# Autodesk Inventor assembly: ASSEMBLY_Y_axis_linear_shaft_mount
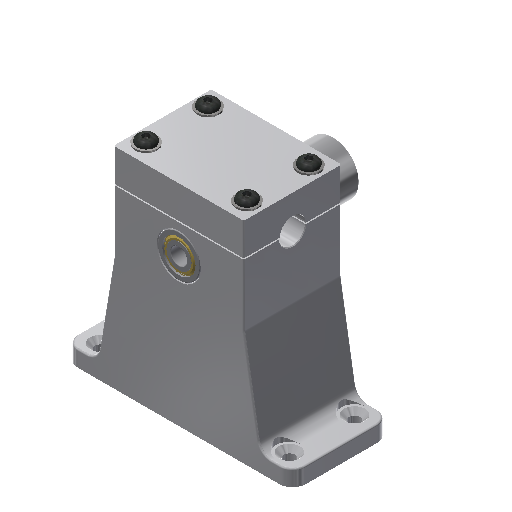
[picture p0: Inventor's stored thumbnail of the model, 512x512]
Saved by Autodesk Inventor 2026.1 (Build 301233000, 233)
## iProperties
Created: 2018-07-31
Part Number: ASSEMBLY_Y_axis_linear_shaft_mount
Document SubType Name: Assembly
Designer: Andrzej
Author: Andrzej
## Documents named in this file (8)
- C:\Users\Andrzej\OneDrive\_DRIVE_SYNCH_FILES\__ BYTECHLAB PROJECTS\MLTDIS - SMD Parts Sorting Machine\MCAD\1_REV1\ASSEMBLY_XY_AXIS_REVA\ASSEMBLY_Y_axis_linear_shaft_mount.iam
- C:\Users\Andrzej\OneDrive\_DRIVE_SYNCH_FILES\__ BYTECHLAB PROJECTS\MLTDIS - SMD Parts Sorting Machine\MCAD\1_REV1\ASSEMBLY_XY_AXIS_REVA\3DP_PLA_Y_axis_linear_shaft_mount_clamp.ipt
- C:\Users\Andrzej\OneDrive\_DRIVE_SYNCH_FILES\__ BYTECHLAB PROJECTS\MLTDIS - SMD Parts Sorting Machine\MCAD\1_REV1\ASSEMBLY_XY_AXIS_REVA\3DP_PLA_Y_axis_linear_shaft_mount.ipt
- C:\Users\Andrzej\OneDrive\_DRIVE_SYNCH_FILES\__ BYTECHLAB PROJECTS\MLTDIS - SMD Parts Sorting Machine\MCAD\1_REV1\__COTS_PARTS\COTS_AST_695HZZ_Bearing.ipt
- C:\Users\Andrzej\OneDrive\_DRIVE_SYNCH_FILES\__ BYTECHLAB PROJECTS\MLTDIS - SMD Parts Sorting Machine\MCAD\1_REV1\__COTS_PARTS\COTS_GENERIC_GT2_20T_Pulley.ipt
- C:\Users\Andrzej\OneDrive\_DRIVE_SYNCH_FILES\__ BYTECHLAB PROJECTS\MLTDIS - SMD Parts Sorting Machine\MCAD\1_REV1\ASSEMBLY_XY_AXIS_REVA\3DP_PLA_Y_axis_drive_shaft_pulley_washer.ipt
- C:\Users\Andrzej\OneDrive\_DRIVE_SYNCH_FILES\__ BYTECHLAB PROJECTS\MLTDIS - SMD Parts Sorting Machine\MCAD\1_REV1\__CONTENT_CENTER_PARTS\en-US\DIN 125-2  A\DIN 125-2 - A 3,2A.ipt
- C:\Users\Andrzej\OneDrive\_DRIVE_SYNCH_FILES\__ BYTECHLAB PROJECTS\MLTDIS - SMD Parts Sorting Machine\MCAD\1_REV1\__CONTENT_CENTER_PARTS\en-US\ISO 7380-1\ISO 7380-1 - M3 x 30.ipt
## Components (14 placed, 7 different names)
1. 3DP_PLA_Y_axis_linear_shaft_mount_clamp:1 — Mate:1, Flush:1, Flush:2, Insert:1, Insert:2, Insert:3, Insert:4
2. 3DP_PLA_Y_axis_linear_shaft_mount:1 — Mate:1, Flush:1, Flush:2, Mate:2, Mate:3, Mate:4, Mate:5, Mate:9
3. COTS_AST_695HZZ_Bearing:1 — Mate:2, Mate:3
4. COTS_AST_695HZZ_Bearing:2 — Mate:4, Mate:5, Mate:6, Mate:7
5. COTS_GENERIC_GT2_20T_Pulley:1 — Mate:8, Mate:9
6. 3DP_PLA_Y_axis_drive_shaft_pulley_washer:1 — Mate:6, Mate:7, Mate:8
7. DIN 125-2 A A 3,2:1 — Insert:1, Insert:5
8. DIN 125-2 A A 3,2:2 — Insert:2, Insert:8
9. DIN 125-2 A A 3,2:3 — Insert:3, Insert:7
10. DIN 125-2 A A 3,2:4 — Insert:4, Insert:6
11. ISO 7380-1 M3 x 30:1 — Insert:5
12. ISO 7380-1 M3 x 30:2 — Insert:6
13. ISO 7380-1 M3 x 30:3 — Insert:7
14. ISO 7380-1 M3 x 30:4 — Insert:8
## Relationships (19: Mate 9, Insert 8, Flush 2)
- Mate:1 (0.4 mm): 3DP_PLA_Y_axis_linear_shaft_mount_clamp:1 ↔ 3DP_PLA_Y_axis_linear_shaft_mount:1
- Flush:1: 3DP_PLA_Y_axis_linear_shaft_mount_clamp:1 ↔ 3DP_PLA_Y_axis_linear_shaft_mount:1
- Flush:2: 3DP_PLA_Y_axis_linear_shaft_mount_clamp:1 ↔ 3DP_PLA_Y_axis_linear_shaft_mount:1
- Mate:2: 3DP_PLA_Y_axis_linear_shaft_mount:1 ↔ COTS_AST_695HZZ_Bearing:1
- Mate:3: 3DP_PLA_Y_axis_linear_shaft_mount:1 ↔ COTS_AST_695HZZ_Bearing:1
- Mate:4: 3DP_PLA_Y_axis_linear_shaft_mount:1 ↔ COTS_AST_695HZZ_Bearing:2
- Mate:5: 3DP_PLA_Y_axis_linear_shaft_mount:1 ↔ COTS_AST_695HZZ_Bearing:2
- Mate:6: COTS_AST_695HZZ_Bearing:2 ↔ 3DP_PLA_Y_axis_drive_shaft_pulley_washer:1
- Mate:7: COTS_AST_695HZZ_Bearing:2 ↔ 3DP_PLA_Y_axis_drive_shaft_pulley_washer:1
- Mate:8: COTS_GENERIC_GT2_20T_Pulley:1 ↔ 3DP_PLA_Y_axis_drive_shaft_pulley_washer:1
- Mate:9: 3DP_PLA_Y_axis_linear_shaft_mount:1 ↔ COTS_GENERIC_GT2_20T_Pulley:1
- Insert:1: 3DP_PLA_Y_axis_linear_shaft_mount_clamp:1 ↔ DIN 125-2 A A 3,2:1
- Insert:2: 3DP_PLA_Y_axis_linear_shaft_mount_clamp:1 ↔ DIN 125-2 A A 3,2:2
- Insert:3: 3DP_PLA_Y_axis_linear_shaft_mount_clamp:1 ↔ DIN 125-2 A A 3,2:3
- Insert:4: 3DP_PLA_Y_axis_linear_shaft_mount_clamp:1 ↔ DIN 125-2 A A 3,2:4
- Insert:5: DIN 125-2 A A 3,2:1 ↔ ISO 7380-1 M3 x 30:1
- Insert:6: DIN 125-2 A A 3,2:4 ↔ ISO 7380-1 M3 x 30:2
- Insert:7: DIN 125-2 A A 3,2:3 ↔ ISO 7380-1 M3 x 30:3
- Insert:8: DIN 125-2 A A 3,2:2 ↔ ISO 7380-1 M3 x 30:4
